# Autodesk Inventor assembly: X-Gantry Assembly for 4040 V1
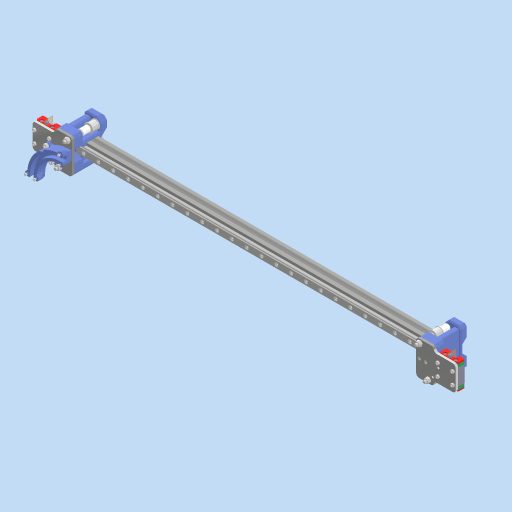
[picture p0: Inventor's stored thumbnail of the model, 512x512]
Saved by Autodesk Inventor 2023.2 (Build 272271000, 271)
## iProperties
Created: 2023-11-20
Part Number: X-Gantry Assembly for 4040 V1
Document SubType Name: Assembly
Designer: Nils Bade
Author: Nils Bade
## Documents named in this file (6)
- C:\Users\nilsb\Documents\Inventor\Projektarbeit-Bade\RatRig_Bade\X-Gantry Assembly for 4040 V2.iam
- X-Gantry Assembly for 4040 V2.iam
- C:\Users\nilsb\Documents\Inventor\Projektarbeit-Bade\RatRig_Standards\V-Slot 2020 - Black - 622mm v1.ipt
- C:\Users\nilsb\Documents\Inventor\Projektarbeit-Bade\RatRig_Standards\MGN12R 600mm 2020 Assembly v2.iam
- C:\Users\nilsb\Documents\Inventor\Projektarbeit-Bade\RatRig_Bade\X-Gantry Joiner Left V2 Assembly.iam
- C:\Users\nilsb\Documents\Inventor\Projektarbeit-Bade\RatRig_Bade\X-Gantry Joiner Right V2 Assembly.iam
## Components (4 placed, 4 different names)
1. V-Slot 2020 - Black - 622mm v1:1 — Passend:29, Fluchtend:31, Passend:30, Passend:31, Fluchtend:32, Passend:32, Fluchtend:33, Passend:33, Passend:34
2. MGN12R 600mm 2020 Assembly v2:1 [sub-assembly] — Passend:29, Fluchtend:31, Passend:30
3. X-Gantry Joiner Left V2 Assembly:1 [sub-assembly] — Passend:31, Fluchtend:32, Passend:32
4. X-Gantry Joiner Right V2 Assembly:1 [sub-assembly] — Fluchtend:33, Passend:33, Passend:34
## Relationships (9: Mate 6, Flush 3)
- Passend:29 [Mate]: V-Slot 2020 - Black - 622mm v1:1 ↔ MGN12R 600mm 2020 Assembly v2:1
- Fluchtend:31 [Flush]: V-Slot 2020 - Black - 622mm v1:1 ↔ MGN12R 600mm 2020 Assembly v2:1
- Passend:30 [Mate]: V-Slot 2020 - Black - 622mm v1:1 ↔ MGN12R 600mm 2020 Assembly v2:1
- Passend:31 [Mate]: V-Slot 2020 - Black - 622mm v1:1 ↔ X-Gantry Joiner Left V2 Assembly:1
- Fluchtend:32 [Flush]: V-Slot 2020 - Black - 622mm v1:1 ↔ X-Gantry Joiner Left V2 Assembly:1
- Passend:32 [Mate]: V-Slot 2020 - Black - 622mm v1:1 ↔ X-Gantry Joiner Left V2 Assembly:1
- Fluchtend:33 [Flush]: V-Slot 2020 - Black - 622mm v1:1 ↔ X-Gantry Joiner Right V2 Assembly:1
- Passend:33 [Mate]: V-Slot 2020 - Black - 622mm v1:1 ↔ X-Gantry Joiner Right V2 Assembly:1
- Passend:34 [Mate]: V-Slot 2020 - Black - 622mm v1:1 ↔ X-Gantry Joiner Right V2 Assembly:1
